# Autodesk Inventor assembly: Glass Door from Laminated Board
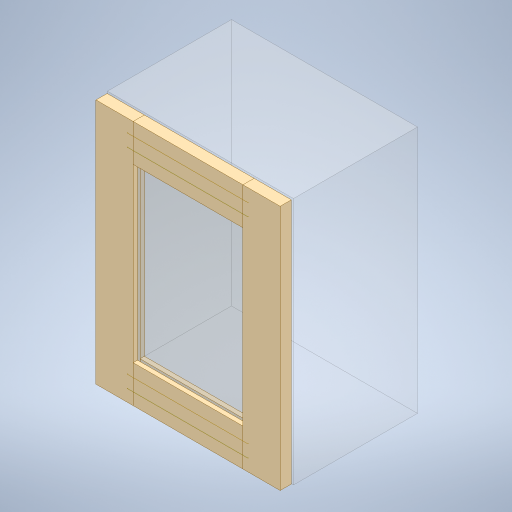
[picture p0: Inventor's stored thumbnail of the model, 512x512]
Saved by Autodesk Inventor 2024 (Build 280153000, 153)
## iProperties
RuleStatus: InUse
Created: 2014-05-07
Part Number: Glass Door from Laminated Board
Document SubType Name: Assembly
Designer: SauliusD
Description: Glass Door from Laminated Board
Author: SauliusD
## Documents named in this file (3)
- C:\W4INV 2024 Design\iBOX LIBRARY\Facades\Glass Door from Laminated Board\Glass Door from Laminated Board.iam
- C:\W4INV 2024 Design\iBOX LIBRARY\Facades\Glass Door from Laminated Board\Glass Door from Laminated Board Skeleton.ipt
- C:\W4INV 2024 Design\iBOX LIBRARY\Facades\Glass Door from Laminated Board\Glass Door from Laminated Board For Gluing.iam
## Components (2 placed, 2 different names)
1. @Skeleton — Flush:4, Flush:5, Flush:6
2. Glass Door from Laminated Board For Gluing:1 [sub-assembly] — Flush:7, Flush:8, Flush:9
## Relationships (6: Flush 6)
- Flush:4: @Skeleton
- Flush:5: @Skeleton
- Flush:6: @Skeleton
- Flush:7: Glass Door from Laminated Board For Gluing:1
- Flush:8: Glass Door from Laminated Board For Gluing:1
- Flush:9: Glass Door from Laminated Board For Gluing:1
## Named parameters: Offset_From_Left = 1.5 mm, Offset_From_Right = 1.5 mm, Offset_From_Top = 1.5 mm, Offset_From_Bottom = 1.5 mm, Panel_Thickness = 18 mm
